# Autodesk Inventor assembly: Flotador
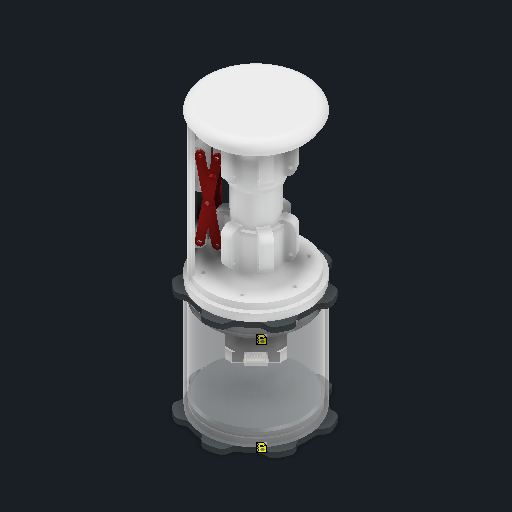
[picture p0: Inventor's stored thumbnail of the model, 512x512]
Saved by Autodesk Inventor 2025.3 (Build 293356030, 356C)
## iProperties
Created: 2024-12-25
Part Number: Flotador
Document SubType Name: Assembly
Designer: Usuario
Author: Usuario
## Documents named in this file (6)
- C:\Users\santa\OneDrive - Universidad de los Andes\Robocol\Flotador\V3\Flotador.iam
- C:\Users\santa\OneDrive - Universidad de los Andes\Robocol\Flotador\V3\Chasis.iam
- C:\Users\santa\OneDrive - Universidad de los Andes\Robocol\Flotador\V3\Expansor.iam
- C:\Users\santa\OneDrive - Universidad de los Andes\Robocol\Flotador\Downloads\17HS4401S Stepper Motor\17HS4401S Stepper Motor_SUB.ipt
- C:\Users\santa\OneDrive - Universidad de los Andes\Robocol\Flotador\Downloads\Flexible Coupler Body\Flexible Coupler Body.ipt
- C:\Users\santa\OneDrive - Universidad de los Andes\Robocol\Flotador\Downloads\lead screw 8mm\lead screw 8mm.ipt
## Components (5 placed, 5 different names)
1. Chasis:1 [sub-assembly] — Nivelación:1, Nivelación:2, Nivelación:3, Rígido:1, Rígido:2
2. Expansor:1 [sub-assembly] — Rígido:1, Coincidencia:21
3. 17HS4401S Stepper Motor_SUB:1 — Rígido:2, De rotación:1
4. Flexible Coupler Body:1 — De rotación:1, Rígido:3
5. lead screw 8mm:1 — Rígido:3, Coincidencia:21
## Relationships (8: Flush 3, WeldJoint 3, RevoluteJoint 1, Mate 1)
- Nivelación:1 [Flush]: Chasis:1
- Nivelación:2 [Flush]: Chasis:1
- Nivelación:3 [Flush]: Chasis:1
- Rígido:1 [WeldJoint]: Chasis:1 ↔ Expansor:1
- Rígido:2 [WeldJoint]: Chasis:1 ↔ 17HS4401S Stepper Motor_SUB:1
- De rotación:1 [RevoluteJoint]: 17HS4401S Stepper Motor_SUB:1 ↔ Flexible Coupler Body:1
- Rígido:3 [WeldJoint]: Flexible Coupler Body:1 ↔ lead screw 8mm:1
- Coincidencia:21 [Mate]: Expansor:1 ↔ lead screw 8mm:1
